# Autodesk Inventor assembly: ASY SLM 0100 frame
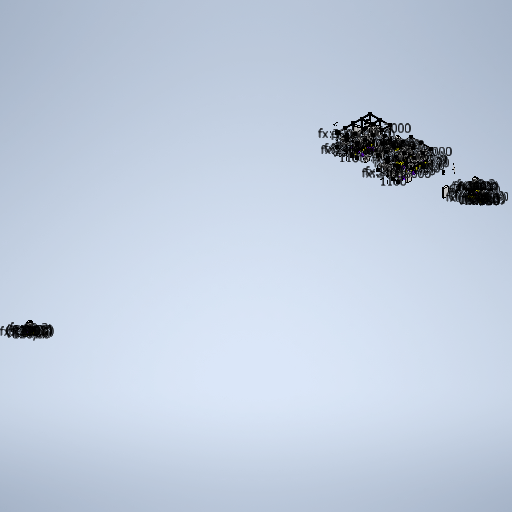
[picture p0: Inventor's stored thumbnail of the model, 512x512]
Saved by Autodesk Inventor 2025 (Build 290162010, 162A)
## iProperties
Created: 2025-12-15
Part Number: ASY SLM 0100 frame
Document SubType Name: Assembly
Designer: admin
Author: admin
## Documents named in this file (13)
- C:\Users\admin\Yandex.Disk\home pc\Inventor\SLM Salemal\ASY SLM 0100 frame.iam
- C:\Users\admin\Yandex.Disk\home pc\Inventor\SLM Salemal\ASY SLM 1600 Filter column D1000.iam
- C:\Users\admin\Yandex.Disk\home pc\Inventor\SLM Salemal\Control box №1.ipt
- C:\Users\admin\Yandex.Disk\home pc\Inventor\SLM Salemal\Control box №2.ipt
- C:\Users\admin\Yandex.Disk\home pc\Inventor\SLM Salemal\Оборудование Инвентор\HY-H H2162–4T.ipt
- C:\Users\admin\Yandex.Disk\home pc\Inventor\SLM Salemal\Оборудование Инвентор\UV-Cleaner ODV-15.ipt
- C:\Users\admin\Yandex.Disk\home pc\Inventor\SLM Salemal\Оборудование Инвентор\Станции дозирования\Coagulant barrel.ipt
- C:\Users\admin\Yandex.Disk\home pc\Inventor\SLM Salemal\Оборудование Инвентор\Станции дозирования\Flocculant barrel.ipt
- C:\Users\admin\Yandex.Disk\home pc\Inventor\SLM Salemal\Оборудование Инвентор\Станции дозирования\GPHN barrel.ipt
- C:\Users\admin\Yandex.Disk\home pc\Inventor\SLM Salemal\Оборудование Инвентор\Станции дозирования\Soda barrel.ipt
- C:\Users\admin\Yandex.Disk\home pc\Inventor\SLM Salemal\Оборудование Инвентор\Вертикальный насос\CDM(F)15-4 FSWP(S_L)C\CDM(F)15-4 FSWP(S_L)C.iam
- C:\Users\admin\Yandex.Disk\home pc\Inventor\SLM Salemal\Оборудование Инвентор\Вертикальный насос\CDM(F)65-2-2 FSWP(S)C\CDM(F)65-2-2 FSWP(S)C.iam
- C:\Users\admin\Yandex.Disk\home pc\Inventor\SLM Salemal\ASY SLM 1110 MAIN FRAME.iam
## Components (59 placed, 12 different names)
1. ASY SLM 1600 Filter column D1000:5 [sub-assembly]
2. ASY SLM 1600 Filter column D1000:6 [sub-assembly]
3. ASY SLM 1600 Filter column D1000:7 [sub-assembly]
4. Control box №1:1
5. Control box №2:1
6. HY-H H2162–4T:1
7. UV-Cleaner ODV-15:1
8. Coagulant barrel:1
9. Flocculant barrel:1
10. GPHN barrel:1
11. Soda barrel:1
12. CDM(F)15-4 FSWP(S_L)C:1 [sub-assembly]
13. CDM(F)65-2-2 FSWP(S)C:1 [sub-assembly]
14. Control box №2:2
15. HY-H H2162–4T:2
16. CDM(F)15-4 FSWP(S_L)C:2 [sub-assembly]
17. CDM(F)65-2-2 FSWP(S)C:2 [sub-assembly]
18. Control box №1:2
19. Control box №1:3
20. UV-Cleaner ODV-15:2
21. ASY SLM 1110 MAIN FRAME:1 [sub-assembly]
22. ASY SLM 1600 Filter column D1000:8 [sub-assembly] — Flush:1, Flush:2, Flush:9, Mate:25, Mate:34
23. ASY SLM 1600 Filter column D1000:9 [sub-assembly]
24. ASY SLM 1600 Filter column D1000:10 [sub-assembly]
25. ASY SLM 1600 Filter column D1000:11 [sub-assembly] — Flush:1, Mate:26, Mate:34
26. ASY SLM 1600 Filter column D1000:12 [sub-assembly] — Flush:3, Mate:21, Flush:7, Mate:22, Flush:8, Flush:9
27. ASY SLM 1600 Filter column D1000:13 [sub-assembly] — Flush:3, Flush:4, Mate:22, Mate:27, Mate:31
28. ASY SLM 1600 Filter column D1000:14 [sub-assembly] — Flush:4, Flush:5, Mate:28, Mate:31, Mate:32
29. Control box №1:4
30. Control box №2:3
31. HY-H H2162–4T:3
32. UV-Cleaner ODV-15:3
33. Coagulant barrel:2
34. Flocculant barrel:2
35. GPHN barrel:2
36. Soda barrel:2
37. CDM(F)15-4 FSWP(S_L)C:3 [sub-assembly]
38. CDM(F)65-2-2 FSWP(S)C:3 [sub-assembly]
39. Control box №2:4
40. HY-H H2162–4T:4
41. CDM(F)15-4 FSWP(S_L)C:4 [sub-assembly]
42. CDM(F)65-2-2 FSWP(S)C:4 [sub-assembly]
43. Control box №1:5
44. Control box №1:6
45. UV-Cleaner ODV-15:4
46. ASY SLM 1110 MAIN FRAME:2 [sub-assembly] — Flush:2, Mate:21, Flush:7, Mate:23, Flush:8, Mate:24, Mate:25, Mate:26, Mate:27, Mate:28, Mate:29, Mate:30
47. ASY SLM 1600 Filter column D1000:15 [sub-assembly] — Flush:5, Flush:6, Mate:29, Mate:32, Mate:33
48. ASY SLM 1600 Filter column D1000:16 [sub-assembly] — Flush:6, Mate:30, Mate:33
49. ASY SLM 1600 Filter column D1000:17 [sub-assembly]
50. Control box №1:7
51. ASY SLM 1600 Filter column D1000:18 [sub-assembly]
52. CDM(F)15-4 FSWP(S_L)C:5 [sub-assembly]
53. ASY SLM 1600 Filter column D1000:20 [sub-assembly]
54. ASY SLM 1600 Filter column D1000:21 [sub-assembly]
55. ASY SLM 1600 Filter column D1000:22 [sub-assembly]
56. ASY SLM 1600 Filter column D1000:23 [sub-assembly]
57. ASY SLM 1600 Filter column D1000:24 [sub-assembly]
58. ASY SLM 1600 Filter column D1000:25 [sub-assembly]
59. ASY SLM 1600 Filter column D1000:26 [sub-assembly]
## Relationships (41: Mate 32, Flush 9)
- [Mate]: ASY SLM 1600 Filter column D1000:5 ↔ ASY SLM 1110 MAIN FRAME:1
- [Mate]: CDM(F)15-4 FSWP(S_L)C:1 ↔ ASY SLM 1110 MAIN FRAME:1
- [Mate]: CDM(F)65-2-2 FSWP(S)C:1 ↔ ASY SLM 1110 MAIN FRAME:1
- [Mate]: Control box №1:1 ↔ ASY SLM 1110 MAIN FRAME:1
- [Mate]: Coagulant barrel:1 ↔ ASY SLM 1110 MAIN FRAME:1
- [Mate]: Flocculant barrel:1 ↔ ASY SLM 1110 MAIN FRAME:1
- [Mate]: GPHN barrel:1 ↔ ASY SLM 1110 MAIN FRAME:1
- [Mate]: Soda barrel:1 ↔ ASY SLM 1110 MAIN FRAME:1
- [Mate]: ASY SLM 1110 MAIN FRAME:1
- [Mate]: ASY SLM 1600 Filter column D1000:8 ↔ ASY SLM 1110 MAIN FRAME:2
- [Mate]: ASY SLM 1600 Filter column D1000:12 ↔ ASY SLM 1110 MAIN FRAME:2
- [Mate]: CDM(F)15-4 FSWP(S_L)C:3 ↔ ASY SLM 1110 MAIN FRAME:2
- [Mate]: CDM(F)65-2-2 FSWP(S)C:3 ↔ ASY SLM 1110 MAIN FRAME:2
- [Mate]: Control box №1:4 ↔ ASY SLM 1110 MAIN FRAME:2
- [Mate]: Coagulant barrel:2 ↔ ASY SLM 1110 MAIN FRAME:2
- [Mate]: Flocculant barrel:2 ↔ ASY SLM 1110 MAIN FRAME:2
- [Mate]: GPHN barrel:2 ↔ ASY SLM 1110 MAIN FRAME:2
- [Mate]: Soda barrel:2 ↔ ASY SLM 1110 MAIN FRAME:2
- Flush:1: ASY SLM 1600 Filter column D1000:8 ↔ ASY SLM 1600 Filter column D1000:11
- Flush:2 (478 mm): ASY SLM 1600 Filter column D1000:8 ↔ ASY SLM 1110 MAIN FRAME:2
- Flush:3: ASY SLM 1600 Filter column D1000:12 ↔ ASY SLM 1600 Filter column D1000:13
- Flush:4: ASY SLM 1600 Filter column D1000:13 ↔ ASY SLM 1600 Filter column D1000:14
- Flush:5: ASY SLM 1600 Filter column D1000:14 ↔ ASY SLM 1600 Filter column D1000:15
- Flush:6: ASY SLM 1600 Filter column D1000:15 ↔ ASY SLM 1600 Filter column D1000:16
- Mate:21: ASY SLM 1600 Filter column D1000:12 ↔ ASY SLM 1110 MAIN FRAME:2
- Flush:7 (600 mm): ASY SLM 1600 Filter column D1000:12 ↔ ASY SLM 1110 MAIN FRAME:2
- Mate:22 (1012 mm): ASY SLM 1600 Filter column D1000:12 ↔ ASY SLM 1600 Filter column D1000:13
- Mate:23: ASY SLM 1110 MAIN FRAME:2
- Flush:8 (478 mm): ASY SLM 1600 Filter column D1000:12 ↔ ASY SLM 1110 MAIN FRAME:2
- Mate:24: ASY SLM 1110 MAIN FRAME:2
- Flush:9 (-500 mm): ASY SLM 1600 Filter column D1000:8 ↔ ASY SLM 1600 Filter column D1000:12
- Mate:25: ASY SLM 1600 Filter column D1000:8 ↔ ASY SLM 1110 MAIN FRAME:2
- Mate:26: ASY SLM 1600 Filter column D1000:11 ↔ ASY SLM 1110 MAIN FRAME:2
- Mate:27: ASY SLM 1600 Filter column D1000:13 ↔ ASY SLM 1110 MAIN FRAME:2
- Mate:28: ASY SLM 1600 Filter column D1000:14 ↔ ASY SLM 1110 MAIN FRAME:2
- Mate:29: ASY SLM 1110 MAIN FRAME:2 ↔ ASY SLM 1600 Filter column D1000:15
- Mate:30: ASY SLM 1110 MAIN FRAME:2 ↔ ASY SLM 1600 Filter column D1000:16
- Mate:31 (1012 mm): ASY SLM 1600 Filter column D1000:13 ↔ ASY SLM 1600 Filter column D1000:14
- Mate:32 (1012 mm): ASY SLM 1600 Filter column D1000:14 ↔ ASY SLM 1600 Filter column D1000:15
- Mate:33 (1012 mm): ASY SLM 1600 Filter column D1000:15 ↔ ASY SLM 1600 Filter column D1000:16
- Mate:34 (1012 mm): ASY SLM 1600 Filter column D1000:8 ↔ ASY SLM 1600 Filter column D1000:11
## Named parameters: d13_d4 = 0 mm, d14_d5 = 0 mm, d15_d6 = 0 mm, d16_d7 = 0 mm, d17_d8 = 0 mm, d18_d9 = 0 mm, d19_d10 = 0 mm, d20_d11 = 0 mm, d21_d1 = 0 mm
